# Autodesk Inventor assembly: BigggWedge1ToothFullTestAssembly
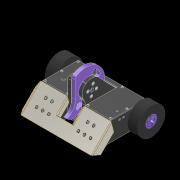
[picture p0: Inventor's stored thumbnail of the model, 180x180]
Saved by Autodesk Inventor 2021 (Build 250183000, 183)
## iProperties
Created: 2020-10-21
Part Number: BigggWedge1ToothFullTestAssembly
Document SubType Name: Assembly
Designer: Esketitttttt
Mass: 465.236 g
Surface Area: 1403.02 cm^2
Volume: 298.301 cm^3
Density: 1.55962 g/cm^3
Author: Esketitttttt
## Documents named in this file (12)
- C:\Users\tandu\Documents\GrabCAD\Insomnia 2020\RRW\BigggWedge1ToothFullTestAssembly.iam
- C:\Users\tandu\Documents\GrabCAD\Insomnia 2020\RRW\Chasis.ipt
- C:\Users\tandu\Documents\GrabCAD\Insomnia 2020\RRW\4-40 x 0.375_ flat head (0.148g).ipt
- C:\Users\tandu\Documents\GrabCAD\Insomnia 2020\RRW\FingerTech_Silver_Spark_223350.ipt
- C:\Users\tandu\Documents\GrabCAD\Insomnia 2020\RRW\Twist_Hub_4mmx075.ipt
- C:\Users\tandu\Documents\GrabCAD\Insomnia 2020\RRW\2_56 Thread_ 3_8 in Long_BUTTON HEAD HEX DRIVE SCREW.ipt
- C:\Users\tandu\Documents\GrabCAD\Insomnia 2020\RRW\power switch _1_.iam
- C:\Users\tandu\Documents\GrabCAD\Insomnia 2020\RRW\2-56 x 0.5_ SHCS (0.146g).ipt
- C:\Users\tandu\Documents\GrabCAD\Insomnia 2020\RRW\2-56 locknut (0.778g) _1_.iam
- C:\Users\tandu\Documents\GrabCAD\Insomnia 2020\RRW\TopPlate.ipt
- C:\Users\tandu\Documents\GrabCAD\Insomnia 2020\RRW\1ToothWeaponAssembly.iam
- C:\Users\tandu\Documents\GrabCAD\Insomnia 2020\RRW\MetalFrontBigggggggWedge.ipt
## Components (39 placed, 11 different names)
1. Chasis:1 — Insert:9, Insert:10, Insert:11, Insert:12, Insert:29, Insert:30, Insert:47, Insert:48, Insert:49, Insert:50, Insert:51, Insert:52, Insert:53, Insert:54, Insert:55, Insert:56, Insert:57, Insert:58, Insert:106, Insert:107, Insert:118, Insert:119
2. FingerTech_Silver_Spark_223350:1 — Insert:9, Insert:10
3. FingerTech_Silver_Spark_223350:2 — Insert:11, Insert:12
4. Twist_Hub_4mmx075:1 — Insert:29
5. Twist_Hub_4mmx075:2 — Insert:30
6. 1ToothWeaponAssembly:1 [sub-assembly] — Insert:47, Insert:48
7. power switch _1_:1 [sub-assembly] — Insert:55, Insert:56, Insert:59, Insert:60
8. TopPlate:1 — Insert:106, Insert:107, Insert:108, Insert:109, Insert:110, Insert:111, Insert:112, Insert:113, Insert:114, Insert:115, Insert:116, Insert:117
9. MetalFrontBigggggggWedge:1 — Insert:118, Insert:119, Insert:120, Insert:121, Insert:122, Insert:123, Insert:124, Insert:125, Insert:126, Insert:127, Insert:128, Insert:129
10. 4-40 x 0.375_ flat head (0.148g):7 — Insert:121
11. 4-40 x 0.375_ flat head (0.148g):8 — Insert:124
12. 4-40 x 0.375_ flat head (0.148g):9 — Insert:122
13. 4-40 x 0.375_ flat head (0.148g):10 — Insert:120
14. 4-40 x 0.375_ flat head (0.148g):11 — Insert:123
15. 4-40 x 0.375_ flat head (0.148g):12 — Insert:127
16. 4-40 x 0.375_ flat head (0.148g):13 — Insert:125
17. 4-40 x 0.375_ flat head (0.148g):14 — Insert:129
18. 4-40 x 0.375_ flat head (0.148g):15 — Insert:126
19. 4-40 x 0.375_ flat head (0.148g):16 — Insert:128
20. 4-40 x 0.375_ flat head (0.148g):1 — Insert:54
21. 4-40 x 0.375_ flat head (0.148g):2 — Insert:52
22. 4-40 x 0.375_ flat head (0.148g):3 — Insert:53
23. 4-40 x 0.375_ flat head (0.148g):4 — Insert:49
24. 4-40 x 0.375_ flat head (0.148g):5 — Insert:50
25. 4-40 x 0.375_ flat head (0.148g):6 — Insert:51
26. 2-56 x 0.5_ SHCS (0.146g):1 — Insert:58
27. 2-56 x 0.5_ SHCS (0.146g):2 — Insert:57
28. 2-56 locknut (0.778g) _1_:1 [sub-assembly] — Insert:60
29. 2-56 locknut (0.778g) _1_:2 [sub-assembly] — Insert:59
30. 2_56 Thread_ 3_8 in Long_BUTTON HEAD HEX DRIVE SCREW:13 — Insert:115
31. 2_56 Thread_ 3_8 in Long_BUTTON HEAD HEX DRIVE SCREW:14 — Insert:110
32. 2_56 Thread_ 3_8 in Long_BUTTON HEAD HEX DRIVE SCREW:15 — Insert:111
33. 2_56 Thread_ 3_8 in Long_BUTTON HEAD HEX DRIVE SCREW:16 — Insert:109
34. 2_56 Thread_ 3_8 in Long_BUTTON HEAD HEX DRIVE SCREW:17 — Insert:112
35. 2_56 Thread_ 3_8 in Long_BUTTON HEAD HEX DRIVE SCREW:18 — Insert:114
36. 2_56 Thread_ 3_8 in Long_BUTTON HEAD HEX DRIVE SCREW:19 — Insert:108
37. 2_56 Thread_ 3_8 in Long_BUTTON HEAD HEX DRIVE SCREW:20 — Insert:117
38. 2_56 Thread_ 3_8 in Long_BUTTON HEAD HEX DRIVE SCREW:21 — Insert:113
39. 2_56 Thread_ 3_8 in Long_BUTTON HEAD HEX DRIVE SCREW:22 — Insert:116
## Relationships (44: Insert 44)
- Insert:9: Chasis:1 ↔ FingerTech_Silver_Spark_223350:1
- Insert:10: Chasis:1 ↔ FingerTech_Silver_Spark_223350:1
- Insert:11: Chasis:1 ↔ FingerTech_Silver_Spark_223350:2
- Insert:12: Chasis:1 ↔ FingerTech_Silver_Spark_223350:2
- Insert:29 (3.81 mm): Chasis:1 ↔ Twist_Hub_4mmx075:1
- Insert:30 (3.81 mm): Chasis:1 ↔ Twist_Hub_4mmx075:2
- Insert:47: Chasis:1 ↔ 1ToothWeaponAssembly:1
- Insert:48: Chasis:1 ↔ 1ToothWeaponAssembly:1
- Insert:49: Chasis:1 ↔ 4-40 x 0.375_ flat head (0.148g):4
- Insert:50: Chasis:1 ↔ 4-40 x 0.375_ flat head (0.148g):5
- Insert:51: Chasis:1 ↔ 4-40 x 0.375_ flat head (0.148g):6
- Insert:52: Chasis:1 ↔ 4-40 x 0.375_ flat head (0.148g):2
- Insert:53: Chasis:1 ↔ 4-40 x 0.375_ flat head (0.148g):3
- Insert:54: Chasis:1 ↔ 4-40 x 0.375_ flat head (0.148g):1
- Insert:55: Chasis:1 ↔ power switch _1_:1
- Insert:56: Chasis:1 ↔ power switch _1_:1
- Insert:57: Chasis:1 ↔ 2-56 x 0.5_ SHCS (0.146g):2
- Insert:58: Chasis:1 ↔ 2-56 x 0.5_ SHCS (0.146g):1
- Insert:59: power switch _1_:1 ↔ 2-56 locknut (0.778g) _1_:2
- Insert:60: power switch _1_:1 ↔ 2-56 locknut (0.778g) _1_:1
- Insert:106: Chasis:1 ↔ TopPlate:1
- Insert:107: Chasis:1 ↔ TopPlate:1
- Insert:108: TopPlate:1 ↔ 2_56 Thread_ 3_8 in Long_BUTTON HEAD HEX DRIVE SCREW:19
- Insert:109: TopPlate:1 ↔ 2_56 Thread_ 3_8 in Long_BUTTON HEAD HEX DRIVE SCREW:16
- Insert:110: TopPlate:1 ↔ 2_56 Thread_ 3_8 in Long_BUTTON HEAD HEX DRIVE SCREW:14
- Insert:111: TopPlate:1 ↔ 2_56 Thread_ 3_8 in Long_BUTTON HEAD HEX DRIVE SCREW:15
- Insert:112: TopPlate:1 ↔ 2_56 Thread_ 3_8 in Long_BUTTON HEAD HEX DRIVE SCREW:17
- Insert:113: TopPlate:1 ↔ 2_56 Thread_ 3_8 in Long_BUTTON HEAD HEX DRIVE SCREW:21
- Insert:114: TopPlate:1 ↔ 2_56 Thread_ 3_8 in Long_BUTTON HEAD HEX DRIVE SCREW:18
- Insert:115: TopPlate:1 ↔ 2_56 Thread_ 3_8 in Long_BUTTON HEAD HEX DRIVE SCREW:13
- Insert:116: TopPlate:1 ↔ 2_56 Thread_ 3_8 in Long_BUTTON HEAD HEX DRIVE SCREW:22
- Insert:117: TopPlate:1 ↔ 2_56 Thread_ 3_8 in Long_BUTTON HEAD HEX DRIVE SCREW:20
- Insert:118: Chasis:1 ↔ MetalFrontBigggggggWedge:1
- Insert:119: Chasis:1 ↔ MetalFrontBigggggggWedge:1
- Insert:120: MetalFrontBigggggggWedge:1 ↔ 4-40 x 0.375_ flat head (0.148g):10
- Insert:121: MetalFrontBigggggggWedge:1 ↔ 4-40 x 0.375_ flat head (0.148g):7
- Insert:122: MetalFrontBigggggggWedge:1 ↔ 4-40 x 0.375_ flat head (0.148g):9
- Insert:123: MetalFrontBigggggggWedge:1 ↔ 4-40 x 0.375_ flat head (0.148g):11
- Insert:124: MetalFrontBigggggggWedge:1 ↔ 4-40 x 0.375_ flat head (0.148g):8
- Insert:125: MetalFrontBigggggggWedge:1 ↔ 4-40 x 0.375_ flat head (0.148g):13
- Insert:126: MetalFrontBigggggggWedge:1 ↔ 4-40 x 0.375_ flat head (0.148g):15
- Insert:127: MetalFrontBigggggggWedge:1 ↔ 4-40 x 0.375_ flat head (0.148g):12
- Insert:128: MetalFrontBigggggggWedge:1 ↔ 4-40 x 0.375_ flat head (0.148g):16
- Insert:129: MetalFrontBigggggggWedge:1 ↔ 4-40 x 0.375_ flat head (0.148g):14
